# Autodesk Inventor assembly: keyboard
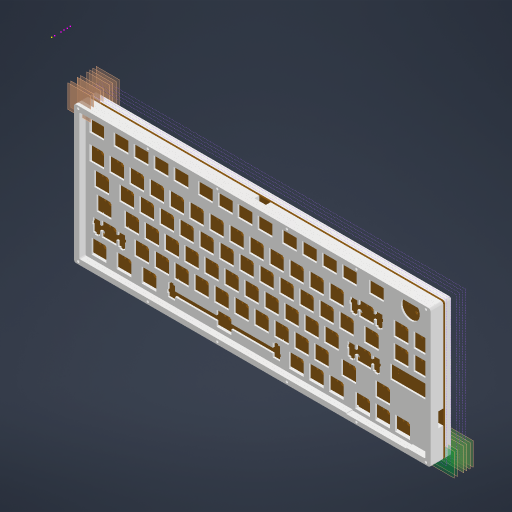
[picture p0: Inventor's stored thumbnail of the model, 512x512]
Saved by Autodesk Inventor 2024.2 (Build 282272000, 272)
## iProperties
Created: 2024-06-20
Part Number: keyboard
Document SubType Name: Assembly
Designer: Moe
Author: Moe
## Documents named in this file (11)
- D:\Code\git\Model-B\case\keyboard.iam
- D:\Code\git\Model-B\case\swplate.ipt
- D:\Code\git\Model-B\case\top-layer.ipt
- D:\Code\git\Model-B\case\open_liner.ipt
- D:\Code\git\Model-B\case\model-b-pcb.ipt
- D:\Code\git\Model-B\case\closed_liner.ipt
- D:\Code\git\Model-B\case\rear_plate.ipt
- D:\Code\git\Model-B\case\foot1.ipt
- D:\Code\git\Model-B\case\foot2.ipt
- D:\Code\git\Model-B\case\foot3.ipt
- D:\Code\git\Model-B\case\foot4.ipt
## Components (11 placed, 10 different names)
1. swplate:1 — Mate:1, Mate:2
2. top-layer:1 — Mate:1, Mate:6
3. open_liner:1 — Mate:2, Mate:3
4. model-b-pcb:1 — Mate:3, Mate:4
5. closed_liner:1 — Mate:4, Mate:5
6. rear_plate:1 — Mate:5, Mate:7
7. top-layer:2 — Mate:6
8. foot1:1 — Mate:7, Mate:8
9. foot2:1 — Mate:8, Mate:9
10. foot3:1 — Mate:9, Mate:10
11. foot4:1 — Mate:10
## Relationships (10: Mate 10)
- Mate:1: swplate:1 ↔ top-layer:1
- Mate:2: swplate:1 ↔ open_liner:1
- Mate:3: open_liner:1 ↔ model-b-pcb:1
- Mate:4: model-b-pcb:1 ↔ closed_liner:1
- Mate:5: closed_liner:1 ↔ rear_plate:1
- Mate:6: top-layer:1 ↔ top-layer:2
- Mate:7: rear_plate:1 ↔ foot1:1
- Mate:8: foot1:1 ↔ foot2:1
- Mate:9: foot2:1 ↔ foot3:1
- Mate:10: foot3:1 ↔ foot4:1
## Named parameters: Finish10_Area = 2020.83, Finish11_Area = 910.719, Finish12_Area = 910.719, Finish13_Area = 910.719, Finish14_Area = 910.719, Finish15_Area = 148.062, Finish16_Area = 640.413, Finish1_Area = 45.1814, Finish2_Area = 278.578, Finish3_Area = 603.709, Finish4_Area = 68.6655, Finish5_Area = 20.7818, Finish6_Area = 66.4595, Finish7_Area = 889.514, Finish8_Area = 1917.96, Finish9_Area = 323.187
note: some values were not read from the file. Shown as the stored number, unit unknown: "Finish10_Area", "Finish11_Area", "Finish12_Area", "Finish13_Area", "Finish14_Area", "Finish15_Area", "Finish16_Area", "Finish1_Area", "Finish2_Area", "Finish3_Area", "Finish4_Area", "Finish5_Area", "Finish6_Area", "Finish7_Area", "Finish8_Area", "Finish9_Area".
